# Autodesk Inventor assembly: Yassembly
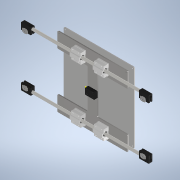
[picture p0: Inventor's stored thumbnail of the model, 180x180]
Saved by Autodesk Inventor 2020.2 (Build 242310000, 310)
## iProperties
Created: 2020-07-30
Part Number: Yassembly
Document SubType Name: Assembly
Designer: JK
Author: JK
## Documents named in this file (11)
- C:\Users\JK\Documents\Inventor\Anet Upgrade\Yassembly.iam
- C:\Users\JK\Documents\Inventor\Anet Upgrade\ycarriage.ipt
- C:\Users\JK\Documents\Inventor\Anet Upgrade\originalbed.ipt
- C:\Users\JK\Documents\Inventor\Anet Upgrade\LinearBearing8mm.iam
- C:\Users\JK\Documents\Inventor\Anet Upgrade\8x380axis.ipt
- C:\Users\JK\Documents\Inventor\Anet Upgrade\YsupportA.ipt
- C:\Users\JK\Documents\Inventor\Anet Upgrade\YsupportB.ipt
- C:\Users\JK\Documents\Inventor\Anet Upgrade\Y Belt Attachment A.ipt
- C:\Users\JK\Documents\Inventor\Anet Upgrade\Y Belt Attachment B.ipt
- C:\Users\JK\Documents\Inventor\Anet Upgrade\M5x15BoltFlatHead.ipt
- C:\Users\JK\Documents\Inventor\Anet Upgrade\T_Slot_Nut_Dropin_3030m5ipt.ipt
## Components (22 placed, 10 different names)
1. ycarriage:1 — Mate:1, Flush:1, Mate:9, Mate:10, Mate:11, Mate:12, Mate:14, Mate:15, Mate:16, Mate:25, Angle:1, Mate:26
2. originalbed:1 — Mate:1, Flush:1, Mate:9
3. LinearBearing8mm:1 [sub-assembly] — Flush:5, Flush:6, Flush:8, Mate:14, Mate:18
4. LinearBearing8mm:2 [sub-assembly] — Flush:5, Mate:16, Flush:9
5. LinearBearing8mm:3 [sub-assembly] — Flush:6, Flush:7, Mate:13, Mate:15, Flush:9
6. LinearBearing8mm:4 [sub-assembly] — Flush:7, Mate:10, Mate:11, Mate:12, Mate:13, Flush:8, Mate:17
7. Wał:1 — Mate:18, Flush:10, Mate:19, Mate:20, Mate:24
8. Wał:2 — Mate:17, Flush:10, Mate:21, Mate:22, Mate:23
9. YsupportA:1 — Mate:19, Mate:20, Flush:11, Flush:12, Flush:13, Mate:31, Angle:4
10. YsupportA:2 — Mate:21, Mate:22, Flush:11, Flush:14, Flush:15, Mate:33
11. YsupportB:1 — Mate:23, Flush:12, Flush:13, Mate:30, Mate:35, Angle:5
12. YsupportB:2 — Mate:24, Flush:14, Flush:15, Mate:32, Angle:2, Mate:40
13. Y Belt Attachment A:1 — Mate:25, Angle:1, Mate:26, Mate:27, Mate:28, Mate:29
14. Y Belt Attachment B:1 — Mate:27, Mate:28, Mate:29
15. M5x15BoltFlatHead:1 — Mate:30, Flush:17, Mate:35, Mate:36
16. M5x15BoltFlatHead:2 — Mate:31, Flush:16, Flush:17, Mate:38
17. M5x15BoltFlatHead:3 — Mate:32, Mate:34, Flush:16, Mate:39
18. M5x15BoltFlatHead:4 — Mate:33, Mate:34, Mate:37
19. T_Slot_Nut_Dropin_3030m5ipt:1 — Mate:36, Angle:5, Flush:18
20. T_Slot_Nut_Dropin_3030m5ipt:2 — Mate:37, Angle:3, Flush:20
21. T_Slot_Nut_Dropin_3030m5ipt:3 — Mate:39, Angle:2, Angle:3, Flush:19, Flush:20, Mate:40
22. T_Slot_Nut_Dropin_3030m5ipt:4 — Mate:38, Angle:4, Flush:18, Flush:19
## Relationships (55: Mate 33, Flush 17, Angle 5)
- Mate:1: ycarriage:1 ↔ originalbed:1
- Flush:1: ycarriage:1 ↔ originalbed:1
- Mate:9 (17 mm): ycarriage:1 ↔ originalbed:1
- Flush:5: LinearBearing8mm:1 ↔ LinearBearing8mm:2
- Flush:6: LinearBearing8mm:1 ↔ LinearBearing8mm:3
- Flush:7: LinearBearing8mm:3 ↔ LinearBearing8mm:4
- Mate:10: ycarriage:1 ↔ LinearBearing8mm:4
- Mate:11: ycarriage:1 ↔ LinearBearing8mm:4
- Mate:12: ycarriage:1 ↔ LinearBearing8mm:4
- Mate:13: LinearBearing8mm:3 ↔ LinearBearing8mm:4
- Flush:8: LinearBearing8mm:1 ↔ LinearBearing8mm:4
- Mate:14: ycarriage:1 ↔ LinearBearing8mm:1
- Mate:15: ycarriage:1 ↔ LinearBearing8mm:3
- Mate:16: ycarriage:1 ↔ LinearBearing8mm:2
- Flush:9: LinearBearing8mm:2 ↔ LinearBearing8mm:3
- Mate:17: LinearBearing8mm:4 ↔ Wał:2
- Mate:18: LinearBearing8mm:1 ↔ Wał:1
- Flush:10: Wał:1 ↔ Wał:2
- Mate:19: Wał:1 ↔ YsupportA:1
- Mate:20: Wał:1 ↔ YsupportA:1
- Mate:21: Wał:2 ↔ YsupportA:2
- Mate:22: Wał:2 ↔ YsupportA:2
- Flush:11: YsupportA:1 ↔ YsupportA:2
- Mate:23: Wał:2 ↔ YsupportB:1
- Flush:12: YsupportA:1 ↔ YsupportB:1
- Flush:13: YsupportA:1 ↔ YsupportB:1
- Mate:24: Wał:1 ↔ YsupportB:2
- Flush:14: YsupportA:2 ↔ YsupportB:2
- Flush:15: YsupportA:2 ↔ YsupportB:2
- Mate:25: ycarriage:1 ↔ Y Belt Attachment A:1
- Angle:1 (0 deg): ycarriage:1 ↔ Y Belt Attachment A:1
- Mate:26: ycarriage:1 ↔ Y Belt Attachment A:1
- Mate:27: Y Belt Attachment A:1 ↔ Y Belt Attachment B:1
- Mate:28: Y Belt Attachment A:1 ↔ Y Belt Attachment B:1
- Mate:29 (0.8 mm): Y Belt Attachment A:1 ↔ Y Belt Attachment B:1
- Mate:30: YsupportB:1 ↔ M5x15BoltFlatHead:1
- Mate:31: YsupportA:1 ↔ M5x15BoltFlatHead:2
- Mate:32: YsupportB:2 ↔ M5x15BoltFlatHead:3
- Mate:33: YsupportA:2 ↔ M5x15BoltFlatHead:4
- Mate:34: M5x15BoltFlatHead:3 ↔ M5x15BoltFlatHead:4
- Flush:16: M5x15BoltFlatHead:2 ↔ M5x15BoltFlatHead:3
- Flush:17: M5x15BoltFlatHead:1 ↔ M5x15BoltFlatHead:2
- Mate:35: YsupportB:1 ↔ M5x15BoltFlatHead:1
- Mate:36: M5x15BoltFlatHead:1 ↔ T_Slot_Nut_Dropin_3030m5ipt:1
- Mate:37: M5x15BoltFlatHead:4 ↔ T_Slot_Nut_Dropin_3030m5ipt:2
- Mate:38: M5x15BoltFlatHead:2 ↔ T_Slot_Nut_Dropin_3030m5ipt:4
- Mate:39: M5x15BoltFlatHead:3 ↔ T_Slot_Nut_Dropin_3030m5ipt:3
- Angle:2 (0 deg): YsupportB:2 ↔ T_Slot_Nut_Dropin_3030m5ipt:3
- Angle:3 (0 deg): T_Slot_Nut_Dropin_3030m5ipt:2 ↔ T_Slot_Nut_Dropin_3030m5ipt:3
- Angle:4 (0 deg): YsupportA:1 ↔ T_Slot_Nut_Dropin_3030m5ipt:4
- Angle:5 (0 deg): YsupportB:1 ↔ T_Slot_Nut_Dropin_3030m5ipt:1
- Flush:18: T_Slot_Nut_Dropin_3030m5ipt:1 ↔ T_Slot_Nut_Dropin_3030m5ipt:4
- Flush:19: T_Slot_Nut_Dropin_3030m5ipt:3 ↔ T_Slot_Nut_Dropin_3030m5ipt:4
- Flush:20: T_Slot_Nut_Dropin_3030m5ipt:2 ↔ T_Slot_Nut_Dropin_3030m5ipt:3
- Mate:40: YsupportB:2 ↔ T_Slot_Nut_Dropin_3030m5ipt:3
